# Autodesk Inventor assembly: ReelAssembly_SBail
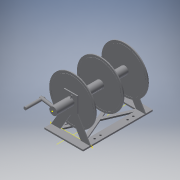
[picture p0: Inventor's stored thumbnail of the model, 180x180]
Saved by Autodesk Inventor 2019 (Build 230136000, 136)
## iProperties
Created: 2019-04-17
Part Number: ReelAssembly_SBail
Document SubType Name: Assembly
Designer: samson.bailor
Author: samson.bailor
## Documents named in this file (9)
- S:\Modern Technology Academy\Bogdziewicz\Student Drop Box\1-Collaboration\47-EDD-2019\Trotline\trotline-reel\src\inventor\ReelAssembly_SBail.iam
- S:\Modern Technology Academy\Bogdziewicz\Student Drop Box\1-Collaboration\47-EDD-2019\Trotline\trotline-reel\src\inventor\Axel_SBail.ipt
- S:\Modern Technology Academy\Bogdziewicz\Student Drop Box\1-Collaboration\47-EDD-2019\Trotline\trotline-reel\src\inventor\Plate.ipt
- S:\Modern Technology Academy\Bogdziewicz\Student Drop Box\1-Collaboration\47-EDD-2019\Trotline\trotline-reel\src\inventor\PlateCenter.ipt
- S:\Modern Technology Academy\Bogdziewicz\Student Drop Box\1-Collaboration\47-EDD-2019\Trotline\trotline-reel\src\inventor\Square Support.ipt
- S:\Modern Technology Academy\Bogdziewicz\Student Drop Box\1-Collaboration\47-EDD-2019\Trotline\trotline-reel\src\inventor\CrankHandle_SBail.ipt
- S:\Modern Technology Academy\Bogdziewicz\Student Drop Box\1-Collaboration\47-EDD-2019\Trotline\trotline-reel\src\inventor\CrankP1_SBail.ipt
- S:\Modern Technology Academy\Bogdziewicz\Student Drop Box\1-Collaboration\47-EDD-2019\Trotline\trotline-reel\src\inventor\CrankP2_SBail.ipt
- S:\Modern Technology Academy\Bogdziewicz\Student Drop Box\1-Collaboration\47-EDD-2019\Trotline\trotline-reel\src\inventor\Pin_SBail.ipt
## Components (9 placed, 8 different names)
1. Axel_SBail:1 — Mate:3, Insert:1, Insert:2, Insert:3, Mate:5, Insert:4
2. PlateCenter:1 — Mate:3
3. Plate:3 — Insert:1
4. Plate:4 — Insert:2
5. Square Support:1 — Insert:3
6. CrankHandle_SBail:1 — Mate:4
7. CrankP2_SBail:1 — Mate:4, Insert:5
8. Pin_SBail:1 — Mate:5
9. CrankP1_SBail:1 — Insert:4, Insert:5
## Relationships (8: Insert 5, Mate 3)
- Mate:3: Axel_SBail:1 ↔ PlateCenter:1
- Insert:1: Axel_SBail:1 ↔ Plate:3
- Insert:2: Axel_SBail:1 ↔ Plate:4
- Insert:3: Axel_SBail:1 ↔ Square Support:1
- Mate:4: CrankHandle_SBail:1 ↔ CrankP2_SBail:1
- Mate:5: Axel_SBail:1 ↔ Pin_SBail:1
- Insert:4: Axel_SBail:1 ↔ CrankP1_SBail:1
- Insert:5: CrankP2_SBail:1 ↔ CrankP1_SBail:1
